# Autodesk Inventor assembly: dummy_drive_train
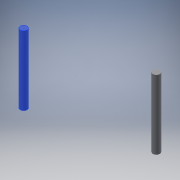
[picture p0: Inventor's stored thumbnail of the model, 180x180]
Saved by Autodesk Inventor 2016 (Build 200138000, 138)
## iProperties
Created: 2016-11-04
Part Number: dummy_drive_train
Document SubType Name: Assembly
Designer: hesaon
Author: hesaon
## Documents named in this file (2)
- D:\documents\SOD-II\cad\dummy_drive_train.iam
- D:\documents\SOD-II\cad\dummy_axle.ipt
## Components (2 placed, 1 different names)
1. dummy_axle:1 — Flush:1
2. dummy_axle:2 — Flush:1
## Relationships (1: Flush 1)
- Flush:1: dummy_axle:1 ↔ dummy_axle:2
